# Autodesk Inventor assembly: crossAssembly
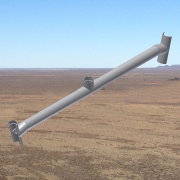
[picture p0: Inventor's stored thumbnail of the model, 180x180]
Saved by Autodesk Inventor 2014 SP1 (Build 180222100, 222)
## iProperties
Created: 2013-12-03
Part Number: crossAssembly
Document SubType Name: Assembly
Designer: Dave
Author: Dave
## Documents named in this file (4)
- C:\Users\Dave\Desktop\hera-cad\surface\crossAssembly.iam
- C:\Users\Dave\Desktop\hera-cad\smallParts\pvc_T_2in.ipt
- C:\Users\Dave\Desktop\hera-cad\surface\cross.ipt
- C:\Users\Dave\Desktop\hera-cad\smallParts\pvc_T_2in_modSplit.ipt
## Components (5 placed, 3 different names)
1. pvc_T_2in:1 — Insert:2, Insert:3
2. cross:1 — Insert:2, Insert:4
3. cross:2 — Insert:3, Insert:5
4. pvc_T_2in_modSplit:1 — Insert:4
5. pvc_T_2in_modSplit:2 — Insert:5
## Relationships (4: Insert 4)
- Insert:2 (-25.4 mm): pvc_T_2in:1 ↔ cross:1
- Insert:3: pvc_T_2in:1 ↔ cross:2
- Insert:4 (-25.4 mm): cross:1 ↔ pvc_T_2in_modSplit:1
- Insert:5 (-25.4 mm): cross:2 ↔ pvc_T_2in_modSplit:2
